# Autodesk Inventor assembly: Chassis - Production Model
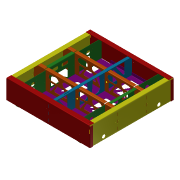
[picture p0: Inventor's stored thumbnail of the model, 180x180]
Saved by Autodesk Inventor 2015 (Build 190159000, 159)
## iProperties
Created: 2015-01-30
Part Number: Chassis - Production Model
Document SubType Name: Assembly
Designer: Peter
Author: Peter
## Documents named in this file (8)
- T:\FILES\FIRST-Team-1719-CAD-Team\2015 Robot CAD\Chassis, Wheels, and Drive Train\Chassis - Production Model\Chassis - Production Model.iam
- T:\FILES\FIRST-Team-1719-CAD-Team\2015 Robot CAD\Chassis, Wheels, and Drive Train\Chassis - Production Model\Base-3.ipt
- T:\FILES\FIRST-Team-1719-CAD-Team\2015 Robot CAD\Chassis, Wheels, and Drive Train\Chassis - Production Model\Front-3.ipt
- T:\FILES\FIRST-Team-1719-CAD-Team\2015 Robot CAD\Chassis, Wheels, and Drive Train\Chassis - Production Model\Outer_Side-3.ipt
- T:\FILES\FIRST-Team-1719-CAD-Team\2015 Robot CAD\Chassis, Wheels, and Drive Train\Chassis - Production Model\CenterBrace-3d.ipt
- T:\FILES\FIRST-Team-1719-CAD-Team\2015 Robot CAD\Chassis, Wheels, and Drive Train\Chassis - Production Model\InnerSide-3-Right.ipt
- T:\FILES\FIRST-Team-1719-CAD-Team\2015 Robot CAD\Chassis, Wheels, and Drive Train\Chassis - Production Model\InnerSide-3.ipt
- T:\FILES\FIRST-Team-1719-CAD-Team\2015 Robot CAD\Chassis, Wheels, and Drive Train\Chassis - Production Model\Brace-3.ipt
## Components (10 placed, 7 different names)
1. Base-3:1 — Mate:8, Mate:9, Mate:10, Mate:11, Mate:12, Mate:13, Mate:14, Mate:15, Mate:16
2. Front-3:1 — Mate:1, Mate:2, Mate:5, Mate:7, Insert:1, Insert:4
3. Outer_Side-3:1 — Mate:1, Mate:3, Mate:4, Mate:5, Insert:1, Insert:2, Mate:21
4. Front-3:2 — Mate:3, Mate:4, Mate:6, Insert:2, Insert:3, Mate:20, Mate:22
5. Outer_Side-3:2 — Mate:2, Mate:6, Mate:7, Insert:3, Insert:4
6. CenterBrace-3d:1 — Mate:14, Mate:15, Mate:16, Flush:1, Mate:22
7. InnerSide-3-Right:1 — Flush:2, Flush:3, Mate:19, Mate:20
8. InnerSide-3:1 — Mate:17, Flush:1, Mate:18, Flush:2, Flush:3
9. Brace-3:1 — Mate:8, Mate:9, Mate:10, Mate:17, Mate:18, Mate:19
10. Brace-3:2 — Mate:11, Mate:12, Mate:13, Mate:21
## Relationships (29: Mate 22, Insert 4, Flush 3)
- Mate:1: Front-3:1 ↔ Outer_Side-3:1
- Mate:2: Front-3:1 ↔ Outer_Side-3:2
- Mate:3: Outer_Side-3:1 ↔ Front-3:2
- Mate:4: Outer_Side-3:1 ↔ Front-3:2
- Mate:5: Front-3:1 ↔ Outer_Side-3:1
- Mate:6: Front-3:2 ↔ Outer_Side-3:2
- Mate:7: Front-3:1 ↔ Outer_Side-3:2
- Insert:1: Front-3:1 ↔ Outer_Side-3:1
- Insert:2: Outer_Side-3:1 ↔ Front-3:2
- Insert:3: Front-3:2 ↔ Outer_Side-3:2
- Insert:4: Front-3:1 ↔ Outer_Side-3:2
- Mate:8: Base-3:1 ↔ Brace-3:1
- Mate:9: Base-3:1 ↔ Brace-3:1
- Mate:10 (0.127 mm): Base-3:1 ↔ Brace-3:1
- Mate:11 (0.127 mm): Base-3:1 ↔ Brace-3:2
- Mate:12 (0.127 mm): Base-3:1 ↔ Brace-3:2
- Mate:13: Base-3:1 ↔ Brace-3:2
- Mate:14 (0.127 mm): Base-3:1 ↔ CenterBrace-3d:1
- Mate:15 (0.127 mm): Base-3:1 ↔ CenterBrace-3d:1
- Mate:16: Base-3:1 ↔ CenterBrace-3d:1
- Mate:17 (0.127 mm): InnerSide-3:1 ↔ Brace-3:1
- Flush:1: CenterBrace-3d:1 ↔ InnerSide-3:1
- Mate:18 (0.7366 mm): InnerSide-3:1 ↔ Brace-3:1
- Flush:2: InnerSide-3-Right:1 ↔ InnerSide-3:1
- Flush:3: InnerSide-3-Right:1 ↔ InnerSide-3:1
- Mate:19: InnerSide-3-Right:1 ↔ Brace-3:1
- Mate:20: Front-3:2 ↔ InnerSide-3-Right:1
- Mate:21: Outer_Side-3:1 ↔ Brace-3:2
- Mate:22 (0.127 mm): Front-3:2 ↔ CenterBrace-3d:1
